# Autodesk Inventor assembly: UpperArmLeft
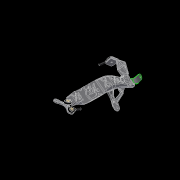
[picture p0: Inventor's stored thumbnail of the model, 180x180]
Saved by Autodesk Inventor 2015 (Build 190159000, 159)
## iProperties
Created: 2014-08-20
Part Number: UpperArmLeft
Document SubType Name: Assembly
Designer: Val
Mass: 413.777 g
Surface Area: 715.953 cm^2
Volume: 168.946 cm^3
Density: 2.44917 g/cm^3
Author: Val
## Documents named in this file (8)
- F:\Exo\Models\3D\UpperArmLeft.iam
- F:\Exo\Models\3D\UpperArmLeft.ipt
- F:\Exo\Models\3D\UpperArmShoulderLeft.ipt
- F:\Exo\Models\3D\UpperArmTricepLeft.ipt
- F:\Exo\Models\3D\External\BearingBody.ipt
- F:\Exo\Models\3D\External\BearingBall.ipt
- F:\Exo\Models\3D\ElbowSubConnectorLeft.ipt
- F:\Exo\Models\3D\UpperArmConnectorLeft.ipt
## Components (11 placed, 7 different names)
1. UpperArmLeft:1 — Mate:49, Mate:94, Mate:95, Mate:96, Mate:97, Mate:98, Mate:99, Mate:100, Mate:105, Mate:106
2. UpperArmShoulderLeft:1 — Mate:49, Mate:52, Mate:53, Angle:1, Mate:94, Mate:95, Mate:96
3. UpperArmTricepLeft:1 — Mate:97, Mate:98, Mate:99
4. BearingBody:1 — Mate:100
5. BearingBody:2
6. BearingBall:1 — Mate:103, Mate:104
7. BearingBall:2 — Mate:101, Mate:102
8. BearingBody:6 — Angle:1
9. BearingBall:6 — Mate:52, Mate:53
10. ElbowSubConnectorLeft:1 — Mate:101, Mate:102, Mate:103, Mate:104
11. UpperArmTwistConnectorLeft:1 — Mate:105, Mate:106
## Relationships (20: Mate 19, Angle 1)
- [Mate]: BearingBody:1 ↔ BearingBall:1
- [Mate]: BearingBody:2 ↔ BearingBall:2
- [Mate]: BearingBody:6 ↔ BearingBall:6
- Mate:49: UpperArmLeft:1 ↔ UpperArmShoulderLeft:1
- Mate:52: UpperArmShoulderLeft:1 ↔ BearingBall:6
- Mate:53: UpperArmShoulderLeft:1 ↔ BearingBall:6
- Angle:1 (0 deg): UpperArmShoulderLeft:1 ↔ BearingBody:6
- Mate:94: UpperArmLeft:1 ↔ UpperArmShoulderLeft:1
- Mate:95: UpperArmLeft:1 ↔ UpperArmShoulderLeft:1
- Mate:96: UpperArmLeft:1 ↔ UpperArmShoulderLeft:1
- Mate:97: UpperArmLeft:1 ↔ UpperArmTricepLeft:1
- Mate:98: UpperArmLeft:1 ↔ UpperArmTricepLeft:1
- Mate:99: UpperArmLeft:1 ↔ UpperArmTricepLeft:1
- Mate:100: UpperArmLeft:1 ↔ BearingBody:1
- Mate:101: BearingBall:2 ↔ ElbowSubConnectorLeft:1
- Mate:102: BearingBall:2 ↔ ElbowSubConnectorLeft:1
- Mate:103: BearingBall:1 ↔ ElbowSubConnectorLeft:1
- Mate:104: BearingBall:1 ↔ ElbowSubConnectorLeft:1
- Mate:105: UpperArmLeft:1 ↔ UpperArmTwistConnectorLeft:1
- Mate:106: UpperArmLeft:1 ↔ UpperArmTwistConnectorLeft:1
## Named parameters: d48_d106 = 0 mm
